# Autodesk Inventor assembly: Cjto para tornillos
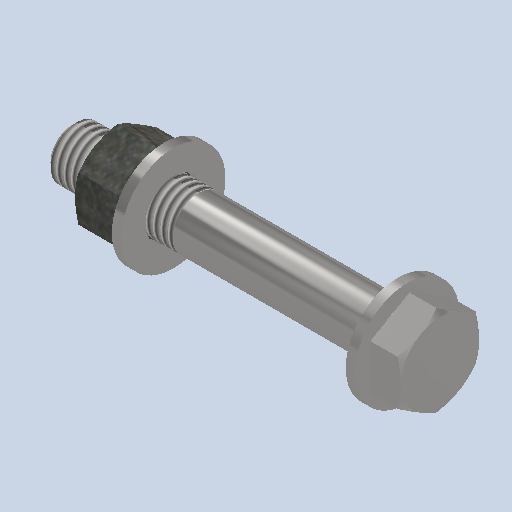
[picture p0: Inventor's stored thumbnail of the model, 512x512]
Saved by Autodesk Inventor 2024 (Build 280153000, 153)
## iProperties
Created: 2026-01-08
Part Number: Cjto para tornillos
Document SubType Name: Assembly
Designer: eduso
Author: eduso
## Documents named in this file (4)
- C:\edusonros_projects\SINFINES_CONRAD\iLogic\Tornilo+tuerca M12x90.iam
- C:\Users\eduso\OneDrive\Documentos\Inventor\Content Center Files\R2024\en-US\ISO 7089\ISO 7089 - 14 - 140 HV(1).ipt
- C:\Users\eduso\OneDrive\Documentos\Inventor\Content Center Files\R2024\en-US\ISO 4014(2)\ISO 4014 - M14 x 90 - ISO.ipt
- C:\Users\eduso\OneDrive\Documentos\Inventor\Content Center Files\R2024\en-US\ISO 4034(2)\ISO 4034 - M14 - ISO.ipt
## Components (4 placed, 3 different names)
1. ISO 7089 14:1 — Insert:1
2. ISO 4014 M14 x 90:1 — Insert:1
3. ISO 7089 14:2 — Insert:2
4. ISO 4034 M14:1 — Insert:2
## Relationships (2: Insert 2)
- Insert:1: ISO 7089 14:1 ↔ ISO 4014 M14 x 90:1
- Insert:2: ISO 7089 14:2 ↔ ISO 4034 M14:1
